# Autodesk Inventor assembly: fc17-067
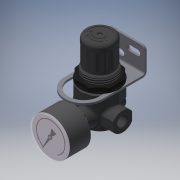
[picture p0: Inventor's stored thumbnail of the model, 180x180]
Saved by Autodesk Inventor 2017.1 (Build 211199000, 199)
## iProperties
Category: Pneumatics
Company: Autodesk Inc.
Created: 2016-12-16
Part Number: fc17-067
Document SubType Name: Assembly
Designer: Autodesk Inc.
Catalog Web Link: http://store.norgren.com/us/en/search.aspx?q=r07-100-rnea
Vendor: Norgren
Description: Main Regulator (assembled)
Author: Autodesk Inc.
Keywords: FIRST Choice
## Documents named in this file (5)
- D:\FIRST\FIRST KOP 2017\FIRST FirstChoice 2017\fc17-067_MountKit.iam
- D:\FIRST\FIRST KOP 2017\FIRST FirstChoice 2017\Parts\Pneumatics_Norgren_R07-100-RNEA.ipt
- D:\FIRST\FIRST KOP 2017\FIRST FirstChoice 2017\Parts\Pneumatics_Norgren_18-025-003_Bracket.ipt
- D:\FIRST\FIRST KOP 2017\FIRST FirstChoice 2017\Parts\Pneumatics_Norgren_18-025-003_Panel Nut.ipt
- D:\FIRST\FIRST KOP 2017\FIRST FirstChoice 2017\Parts\Pneu_Norgren_18-013-212.iam
## Components (4 placed, 4 different names)
1. Pneumatics_Norgren_R07-100-RNEA:1 — Mate:1, Mate:2, Mate:3, Insert:1
2. Pneumatics_Norgren_18-025-003_Bracket:1 — Mate:1, Mate:2, Mate:4
3. Pneumatics_Norgren_18-025-003_Panel Nut:1 — Mate:3, Mate:4
4. Pneu_Norgren_18-013-212:1 [sub-assembly] — Insert:1
## Relationships (5: Mate 4, Insert 1)
- Mate:1: Pneumatics_Norgren_R07-100-RNEA:1 ↔ Pneumatics_Norgren_18-025-003_Bracket:1
- Mate:2: Pneumatics_Norgren_R07-100-RNEA:1 ↔ Pneumatics_Norgren_18-025-003_Bracket:1
- Mate:3: Pneumatics_Norgren_R07-100-RNEA:1 ↔ Pneumatics_Norgren_18-025-003_Panel Nut:1
- Mate:4: Pneumatics_Norgren_18-025-003_Bracket:1 ↔ Pneumatics_Norgren_18-025-003_Panel Nut:1
- Insert:1: Pneumatics_Norgren_R07-100-RNEA:1 ↔ Pneu_Norgren_18-013-212:1
